# Autodesk Inventor assembly: assembly_support
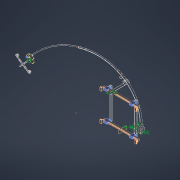
[picture p0: Inventor's stored thumbnail of the model, 180x180]
Saved by Autodesk Inventor 2021 (Build 250183000, 183)
## iProperties
Created: 2021-05-11
Part Number: assembly_support
Document SubType Name: Assembly
Designer: Watchdog
Mass: 54004 g
Surface Area: 34045.7 cm^2
Volume: 9603.57 cm^3
Density: 5.62332 g/cm^3
Author: Watchdog
## Documents named in this file (8)
- C:\Users\Watchdog\OneDrive - Flinders\Advn Mech Design Shared\6_Development\2_Design\inventor\support\assembly_support.iam
- C:\Users\Watchdog\OneDrive - Flinders\Advn Mech Design Shared\6_Development\2_Design\inventor\support\roof_bar\ext_roof bar assembly.iam
- C:\Users\Watchdog\OneDrive - Flinders\Advn Mech Design Shared\6_Development\2_Design\inventor\connection\assembly_connector.iam
- C:\Users\Watchdog\OneDrive - Flinders\Advn Mech Design Shared\6_Development\2_Design\inventor\assembly_hoop.iam
- C:\Users\Watchdog\OneDrive - Flinders\Advn Mech Design Shared\6_Development\2_Design\inventor\support\support_frame_x.ipt
- C:\Users\Watchdog\OneDrive - Flinders\Advn Mech Design Shared\6_Development\2_Design\inventor\rack_pinion\adjust_sheet.ipt
- C:\Users\Watchdog\OneDrive - Flinders\Advn Mech Design Shared\6_Development\2_Design\inventor\support\support_basePart_truss.ipt
- C:\Users\Watchdog\OneDrive - Flinders\Advn Mech Design Shared\6_Development\2_Design\inventor\support\support_frame_z.ipt
## Components (11 placed, 7 different names)
1. ext_roof bar assembly:1 [sub-assembly] — Flush:6, Flush:7, Flush:8, Mate:39, Mate:40, Mate:51
2. ext_roof bar assembly:2 [sub-assembly] — Flush:3, Flush:4, Flush:5, Flush:6, Flush:7, Flush:8, Flush:9, Mate:11, Mate:53, Mate:61
3. assembly_connector:1 [sub-assembly] — Flush:9, Mate:11, Flush:10, Mate:58, Mate:60
4. assembly_connector:2 [sub-assembly] — Mate:39, Mate:40, Flush:10, Mate:59
5. assembly_connector:3 [sub-assembly] — Mate:51, Mate:54, Mate:57, Flush:11
6. assembly_connector:4 [sub-assembly] — Mate:53, Mate:56, Flush:11, Mate:61
7. assembly_hoop:1 [sub-assembly] — Mate:58, Mate:59, Mate:60, Mate:62, Mate:65
8. support_frame_x:1 — Mate:33, Mate:34, Mate:54, Mate:56, Mate:57
9. adjust_sheet:1 — Mate:46, Mate:47, Mate:48, Mate:62, Mate:65
10. support_basePart_truss:1 — Mate:33, Mate:34, Mate:36, Mate:63, Mate:64
11. support_frame_z:1 — Mate:36, Mate:46, Mate:47, Mate:48, Mate:63, Mate:64
## Relationships (31: Mate 22, Flush 9)
- Flush:3: ext_roof bar assembly:2
- Flush:4: ext_roof bar assembly:2
- Flush:5: ext_roof bar assembly:2
- Flush:6 (900 mm): ext_roof bar assembly:1 ↔ ext_roof bar assembly:2
- Flush:7: ext_roof bar assembly:1 ↔ ext_roof bar assembly:2
- Flush:8: ext_roof bar assembly:1 ↔ ext_roof bar assembly:2
- Flush:9: ext_roof bar assembly:2 ↔ assembly_connector:1
- Mate:11: ext_roof bar assembly:2 ↔ assembly_connector:1
- Mate:33: support_frame_x:1 ↔ support_basePart_truss:1
- Mate:34: support_frame_x:1 ↔ support_basePart_truss:1
- Mate:36: support_basePart_truss:1 ↔ support_frame_z:1
- Mate:39: ext_roof bar assembly:1 ↔ assembly_connector:2
- Mate:40: ext_roof bar assembly:1 ↔ assembly_connector:2
- Mate:46: adjust_sheet:1 ↔ support_frame_z:1
- Mate:47: adjust_sheet:1 ↔ support_frame_z:1
- Mate:48: adjust_sheet:1 ↔ support_frame_z:1
- Mate:51: ext_roof bar assembly:1 ↔ assembly_connector:3
- Mate:53: ext_roof bar assembly:2 ↔ assembly_connector:4
- Mate:54: assembly_connector:3 ↔ support_frame_x:1
- Mate:56: assembly_connector:4 ↔ support_frame_x:1
- Mate:57: assembly_connector:3 ↔ support_frame_x:1
- Flush:10: assembly_connector:1 ↔ assembly_connector:2
- Mate:58: assembly_connector:1 ↔ assembly_hoop:1
- Mate:59: assembly_connector:2 ↔ assembly_hoop:1
- Mate:60: assembly_connector:1 ↔ assembly_hoop:1
- Flush:11: assembly_connector:3 ↔ assembly_connector:4
- Mate:61: ext_roof bar assembly:2 ↔ assembly_connector:4
- Mate:62: assembly_hoop:1 ↔ adjust_sheet:1
- Mate:63: support_basePart_truss:1 ↔ support_frame_z:1
- Mate:64: support_basePart_truss:1 ↔ support_frame_z:1
- Mate:65: assembly_hoop:1 ↔ adjust_sheet:1
